# Autodesk Inventor assembly: stalp
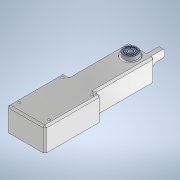
[picture p0: Inventor's stored thumbnail of the model, 180x180]
Saved by Autodesk Inventor 2022 (Build 260153000, 153)
## iProperties
Created: 2022-03-04
Part Number: stalp
Document SubType Name: Assembly
Designer: Oana
Author: Oana
## Documents named in this file (3)
- C:\Users\alexo\Documents\Inventor\Scanner3D\infoeducatia 2022\proiectare\stalp\stalp.iam
- C:\Users\alexo\Documents\Inventor\Scanner3D\infoeducatia 2022\proiectare\stalp\stalp.ipt
- C:\Users\alexo\Documents\Inventor\Scanner3D\Rulment.ipt
## Components (3 placed, 2 different names)
1. stalp:1 — Rigid:3, Flush:1, Mate:1, Rigid:4
2. Rulment:1 — Rigid:3
3. Rulment:2 — Flush:1, Mate:1, Rigid:4
## Relationships (4: WeldJoint 2, Flush 1, Mate 1)
- Rigid:3 [WeldJoint]: stalp:1 ↔ Rulment:1
- Flush:1: stalp:1 ↔ Rulment:2
- Mate:1: stalp:1 ↔ Rulment:2
- Rigid:4 [WeldJoint]: stalp:1 ↔ Rulment:2
